# Autodesk Inventor assembly: 000-ballhand-v2
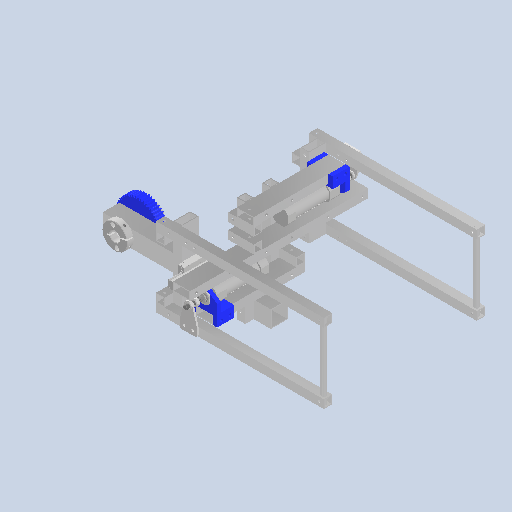
[picture p0: Inventor's stored thumbnail of the model, 512x512]
Saved by Autodesk Inventor 2025.1 (Build 291241000, 241)
## iProperties
Created: 2024-03-16
Part Number: 000-ballhand-v2
Document SubType Name: Assembly
Designer: haruy
Author: haruy
## Documents named in this file (9)
- C:\Users\haruy\Documents\ロボコン\NHK2025\cad\nagahisa\dribl\R2-Rzvector\000-ballhand-v2.iam
- C:\Users\haruy\Documents\ロボコン\NHK2025\cad\nagahisa\dribl\R2-Rzvector\ballhand-v2-ASP-Base.ipt
- C:\Users\haruy\Documents\ロボコン\NHK2025\cad\nagahisa\dribl\R2-Rzvector\ballhand-v2-ASP-H.ipt
- C:\Users\haruy\Documents\ロボコン\NHK2025\cad\nagahisa\dribl\R2-Rzvector\SSEBZ-MX10-55.iam
- C:\Users\haruy\Documents\ロボコン\NHK2025\cad\nagahisa\dribl\R2-Rzvector\ballhand-v2-Plate-H-Air-F.ipt
- C:\Users\haruy\Documents\ロボコン\NHK2025\cad\nagahisa\dribl\R2-Rzvector\ballhand-v2-3DP-Air-F.ipt
- C:\Users\haruy\Documents\ロボコン\NHK2025\cad\nagahisa\dribl\R2-Rzvector\CDJ2B16-15Z-B(0_1_0).iam
- C:\Users\haruy\Documents\ロボコン\NHK2025\cad\nagahisa\dribl\R2-Rzvector\平歯車1.iam
- C:\Users\haruy\Documents\ロボコン\NHK2025\cad\nagahisa\dribl\R2-Rzvector\SSCSM12-8.iam
## Components (14 placed, 8 different names)
1. ballhand-v2-ASP-Base:1 — 挿入:1, 挿入:2, 挿入:3, 挿入:4, 挿入:13, 挿入:14, 挿入:15, 挿入:18, 挿入:19, 挿入:22, 挿入:23
2. ballhand-v2-ASP-H:1 — 挿入:5, 挿入:6, 挿入:9, 挿入:10
3. ballhand-v2-ASP-H:2 — 挿入:7, 挿入:8, 挿入:11, 挿入:12
4. SSEBZ-MX10-55:1 [sub-assembly] — 挿入:1, 挿入:2, 挿入:5, 挿入:6
5. SSEBZ-MX10-55:2 [sub-assembly] — 挿入:3, 挿入:4, 挿入:7, 挿入:8
6. ballhand-v2-Plate-H-Air-F:1 — 挿入:9, 挿入:10, 挿入:20
7. ballhand-v2-Plate-H-Air-F:2 — 挿入:11, 挿入:12, 挿入:21
8. ballhand-v2-3DP-Air-F:1 — 挿入:13, 挿入:16, 挿入:18, 挿入:19
9. ballhand-v2-3DP-Air-F:2 — 挿入:14, 挿入:15, 挿入:17
10. CDJ2B16-15Z-B(0_1_0):1 [sub-assembly] — 挿入:16, 挿入:20
11. CDJ2B16-15Z-B(0_1_0):2 [sub-assembly] — 挿入:17, 挿入:21
12. 平歯車:1 [sub-assembly] — 挿入:22, 挿入:24
13. SSCSM12-8:1 [sub-assembly] — 挿入:23
14. SSCSM12-8:2 [sub-assembly] — 挿入:24
## Relationships (24: Insert 24)
- 挿入:1 [Insert]: ballhand-v2-ASP-Base:1 ↔ SSEBZ-MX10-55:1
- 挿入:2 [Insert]: ballhand-v2-ASP-Base:1 ↔ SSEBZ-MX10-55:1
- 挿入:3 [Insert]: ballhand-v2-ASP-Base:1 ↔ SSEBZ-MX10-55:2
- 挿入:4 [Insert]: ballhand-v2-ASP-Base:1 ↔ SSEBZ-MX10-55:2
- 挿入:5 [Insert]: ballhand-v2-ASP-H:1 ↔ SSEBZ-MX10-55:1
- 挿入:6 [Insert]: ballhand-v2-ASP-H:1 ↔ SSEBZ-MX10-55:1
- 挿入:7 [Insert]: ballhand-v2-ASP-H:2 ↔ SSEBZ-MX10-55:2
- 挿入:8 [Insert]: ballhand-v2-ASP-H:2 ↔ SSEBZ-MX10-55:2
- 挿入:9 [Insert]: ballhand-v2-ASP-H:1 ↔ ballhand-v2-Plate-H-Air-F:1
- 挿入:10 [Insert]: ballhand-v2-ASP-H:1 ↔ ballhand-v2-Plate-H-Air-F:1
- 挿入:11 [Insert]: ballhand-v2-ASP-H:2 ↔ ballhand-v2-Plate-H-Air-F:2
- 挿入:12 [Insert]: ballhand-v2-ASP-H:2 ↔ ballhand-v2-Plate-H-Air-F:2
- 挿入:13 [Insert]: ballhand-v2-ASP-Base:1 ↔ ballhand-v2-3DP-Air-F:1
- 挿入:14 [Insert]: ballhand-v2-ASP-Base:1 ↔ ballhand-v2-3DP-Air-F:2
- 挿入:15 [Insert]: ballhand-v2-ASP-Base:1 ↔ ballhand-v2-3DP-Air-F:2
- 挿入:16 [Insert]: ballhand-v2-3DP-Air-F:1 ↔ CDJ2B16-15Z-B(0_1_0):1
- 挿入:17 [Insert]: ballhand-v2-3DP-Air-F:2 ↔ CDJ2B16-15Z-B(0_1_0):2
- 挿入:18 [Insert]: ballhand-v2-ASP-Base:1 ↔ ballhand-v2-3DP-Air-F:1
- 挿入:19 [Insert]: ballhand-v2-ASP-Base:1 ↔ ballhand-v2-3DP-Air-F:1
- 挿入:20 [Insert] (-4 mm): ballhand-v2-Plate-H-Air-F:1 ↔ CDJ2B16-15Z-B(0_1_0):1
- 挿入:21 [Insert] (-4 mm): ballhand-v2-Plate-H-Air-F:2 ↔ CDJ2B16-15Z-B(0_1_0):2
- 挿入:22 [Insert]: ballhand-v2-ASP-Base:1 ↔ 平歯車:1
- 挿入:23 [Insert]: ballhand-v2-ASP-Base:1 ↔ SSCSM12-8:1
- 挿入:24 [Insert]: 平歯車:1 ↔ SSCSM12-8:2
